# Autodesk Inventor assembly: LargeFinderEyepieces
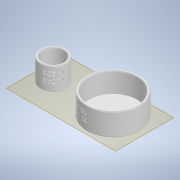
[picture p0: Inventor's stored thumbnail of the model, 180x180]
Saved by Autodesk Inventor 2021.1 (Build 251245000, 245)
## iProperties
Created: 2020-09-27
Part Number: LargeFinderEyepieces
Document SubType Name: Assembly
Designer: robst
Author: robst
## Documents named in this file (3)
- C:\git\CAD-Development\robSteele\TelescopeProjects\LensCovers\LargeFinderEyepieces.iam
- C:\git\CAD-Development\robSteele\TelescopeProjects\LensCovers\LargeFinderEyePieceCover.ipt
- C:\git\CAD-Development\robSteele\TelescopeProjects\LensCovers\LargeFinderObjectiveCover.ipt
## Components (2 placed, 2 different names)
1. LargeFinderEyePieceCover:1 — Mate:1, Flush:1, Flush:2
2. LargeFinderObjectiveCover:1 — Mate:2, Mate:3, Mate:4
## Relationships (6: Mate 4, Flush 2)
- Mate:1: LargeFinderEyePieceCover:1
- Flush:1: LargeFinderEyePieceCover:1
- Flush:2: LargeFinderEyePieceCover:1
- Mate:2: LargeFinderObjectiveCover:1
- Mate:3 (76.2 mm): LargeFinderObjectiveCover:1
- Mate:4: LargeFinderObjectiveCover:1
